# Autodesk Inventor assembly: 19th_0806_04
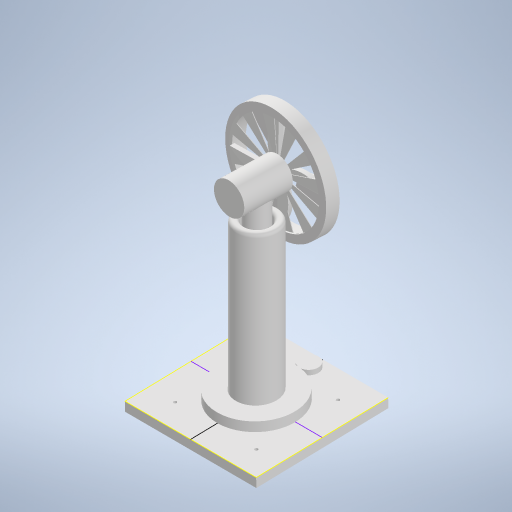
[picture p0: Inventor's stored thumbnail of the model, 512x512]
Saved by Autodesk Inventor 2024 (Build 280153000, 153)
## iProperties
Created: 2024-08-06
Part Number: 19th_0806_04
Document SubType Name: Assembly
Designer: chlqj
Author: chlqj
## Documents named in this file (6)
- C:\Users\chlqj\Documents\19th_0806_04.iam
- C:\Users\chlqj\Documents\fan_num1.ipt
- C:\Users\chlqj\Documents\fan_num2.ipt
- C:\Users\chlqj\Documents\fan_num3.ipt
- C:\Users\chlqj\Documents\fan_num4_1.ipt
- C:\Users\chlqj\Documents\fan_num5_1.ipt
## Components (5 placed, 5 different names)
1. fan_num1:1 — 메이트:1, 메이트:3
2. fan_num2:1 — 메이트:1, 메이트:3
3. fan_num3:1 — 메이트:2, 메이트:4
4. fan_num4_1:1 — 메이트:2
5. fan_num5_1:1 — 메이트:4
## Relationships (4: Mate 4)
- 메이트:1 [Mate]: fan_num1:1 ↔ fan_num2:1
- 메이트:2 [Mate]: fan_num3:1 ↔ fan_num4_1:1
- 메이트:3 [Mate]: fan_num1:1 ↔ fan_num2:1
- 메이트:4 [Mate]: fan_num3:1 ↔ fan_num5_1:1
